# Autodesk Inventor assembly: 简单模型
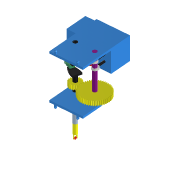
[picture p0: Inventor's stored thumbnail of the model, 180x180]
Saved by Autodesk Inventor 2022 (Build 260153000, 153)
## iProperties
Created: 2023-02-22
Part Number: 简单模型
Document SubType Name: Assembly
Designer: 李承轩
d38: 20.00 deg
Author: 李承轩
## Documents named in this file (14)
- C:\Users\Lzy18\Desktop\发动机模型\发动机模型\简单模型.iam
- C:\Users\Lzy18\Desktop\发动机模型\发动机模型\支撑板1.ipt
- C:\Users\Lzy18\Desktop\发动机模型\发动机模型\动力传输1\设计加速器\正齿轮14.ipt
- C:\Users\Lzy18\Desktop\发动机模型\发动机模型\动力传输1\设计加速器\正齿轮24.ipt
- C:\Users\Lzy18\Desktop\发动机模型\发动机模型\曲轴.ipt
- C:\Users\Lzy18\Desktop\发动机模型\发动机模型\连杆.ipt
- C:\Users\Lzy18\Desktop\发动机模型\发动机模型\连接下环.ipt
- C:\Users\Lzy18\Desktop\发动机模型\发动机模型\主体.ipt
- C:\Users\Lzy18\Desktop\发动机模型\发动机模型\活塞.ipt
- C:\Users\Lzy18\Desktop\发动机模型\发动机模型\轴2.ipt
- C:\Users\Lzy18\Desktop\发动机模型\发动机模型\活塞顶杆.iam
- C:\Users\Lzy18\Desktop\发动机模型\发动机模型\花键.iam
- C:\Users\Lzy18\Desktop\发动机模型\发动机模型\万向节块.ipt
- C:\Users\Lzy18\Desktop\发动机模型\发动机模型\盘式凸轮1.ipt
## Components (16 placed, 13 different names)
1. 支撑板1:1 — 插入:1, 插入:2, 角度:2, 角度:4
2. 正齿轮1:1 — 配合:1, 表面齐平:1, 角度:1, 转动:1, 角度:4
3. 正齿轮2:1 — 插入:2, 转动:1, 配合:9
4. 曲轴:1 — 配合:1, 表面齐平:1, 插入:1, 角度:1, 配合:2, 表面齐平:2, 插入:5, 插入:7
5. 连杆:1 — 插入:3, 插入:4, 配合:2, 表面齐平:2, 配合:4
6. 连接下环:1 — 插入:3, 插入:4
7. 主体:1 — 插入:5, 角度:2, 配合:3, 插入:6, 配合:11, 配合:13
8. 活塞:1 — 配合:3, 配合:4
9. 轴2:1 — 插入:6, 配合:9, 插入:8, 插入:9
10. 活塞顶杆:1 [sub-assembly] — 配合:11, 配合:20, 过渡:1
11. 活塞顶杆:2 [sub-assembly] — 配合:13, 配合:19, 相切:2
12. 花键:1 [sub-assembly] — 插入:7, 配合:15, 配合:16
13. 万向节块:1 — 配合:15, 配合:16, 配合:17, 配合:18
14. 花键:2 [sub-assembly] — 配合:17, 配合:18
15. 盘式凸轮:1 — 插入:8, 配合:19, 相切:2
16. 盘式凸轮:2 — 插入:9, 配合:20, 过渡:1
## Relationships (30: Mate 13, Insert 9, Angle 3, Flush 2, RelateRotation 1, Tangent 1, Transitional 1)
- 配合:1 [Mate]: 正齿轮1:1 ↔ 曲轴:1
- 表面齐平:1 [Flush] (60 mm): 正齿轮1:1 ↔ 曲轴:1
- 插入:1 [Insert]: 支撑板1:1 ↔ 曲轴:1
- 角度:1 [Angle] (0 deg): 正齿轮1:1 ↔ 曲轴:1
- 插入:2 [Insert] (40 mm): 支撑板1:1 ↔ 正齿轮2:1
- 转动:1 [RelateRotation] (2.5 ul): 正齿轮1:1 ↔ 正齿轮2:1
- 插入:3 [Insert]: 连杆:1 ↔ 连接下环:1
- 插入:4 [Insert]: 连杆:1 ↔ 连接下环:1
- 配合:2 [Mate]: 曲轴:1 ↔ 连杆:1
- 表面齐平:2 [Flush]: 曲轴:1 ↔ 连杆:1
- 插入:5 [Insert]: 曲轴:1 ↔ 主体:1
- 角度:2 [Angle] (0 deg): 支撑板1:1 ↔ 主体:1
- 配合:3 [Mate]: 主体:1 ↔ 活塞:1
- 配合:4 [Mate]: 连杆:1 ↔ 活塞:1
- 插入:6 [Insert]: 主体:1 ↔ 轴2:1
- 配合:9 [Mate]: 正齿轮2:1 ↔ 轴2:1
- 配合:11 [Mate]: 主体:1 ↔ 活塞顶杆:1
- 配合:13 [Mate]: 主体:1 ↔ 活塞顶杆:2
- 插入:7 [Insert]: 曲轴:1 ↔ 花键:1
- 配合:15 [Mate]: 花键:1 ↔ 万向节块:1
- 配合:16 [Mate]: 花键:1 ↔ 万向节块:1
- 配合:17 [Mate]: 万向节块:1 ↔ 花键:2
- 配合:18 [Mate]: 万向节块:1 ↔ 花键:2
- 角度:4 [Angle]: 支撑板1:1 ↔ 正齿轮1:1
- 插入:8 [Insert] (70 mm): 轴2:1 ↔ 盘式凸轮:1
- 插入:9 [Insert] (-150 mm): 轴2:1 ↔ 盘式凸轮:2
- 配合:19 [Mate]: 活塞顶杆:2 ↔ 盘式凸轮:1
- 配合:20 [Mate]: 活塞顶杆:1 ↔ 盘式凸轮:2
- 相切:2 [Tangent]: 活塞顶杆:2 ↔ 盘式凸轮:1
- 过渡:1 [Transitional]: 活塞顶杆:1 ↔ 盘式凸轮:2
